# Autodesk Inventor assembly: Rpboticarm
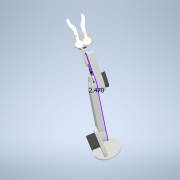
[picture p0: Inventor's stored thumbnail of the model, 180x180]
Saved by Autodesk Inventor 2020 (Build 240168000, 168)
## iProperties
Created: 2020-07-21
Part Number: Rpboticarm
Document SubType Name: Assembly
Designer: Kelvin
Mass: 414.619 g
Surface Area: 1250.55 cm^2
Volume: 414.619 cm^3
Density: 1 g/cm^3
Author: Kelvin
## Documents named in this file (7)
- C:\Users\Kelvin\Desktop\arm\Arm_v2.iam
- C:\Users\Kelvin\Documents\basestand.ipt
- C:\Users\Kelvin\Documents\MG996R_smotor.iam
- C:\Users\Kelvin\Documents\shoulder.ipt
- C:\Users\Kelvin\Documents\arm.ipt
- C:\Users\Kelvin\Desktop\arm\claw.iam
- C:\Users\Kelvin\Desktop\arm\Microservo.0002.iam
## Components (7 placed, 6 different names)
1. basestand:1 — Mate:1, Mate:2
2. shoulder:1 — Mate:3
3. arm:1
4. MG996R_smotor:1 [sub-assembly] — Mate:1, Mate:2, Mate:3
5. MG996R_smotor:2 [sub-assembly]
6. claw:1 [sub-assembly]
7. Microservo.0002:1 [sub-assembly]
## Relationships (3: Mate 3)
- Mate:1: basestand:1 ↔ MG996R_smotor:1
- Mate:2: basestand:1 ↔ MG996R_smotor:1
- Mate:3 (12.7 mm): shoulder:1 ↔ MG996R_smotor:1
